# Autodesk Inventor assembly: 總組合圖
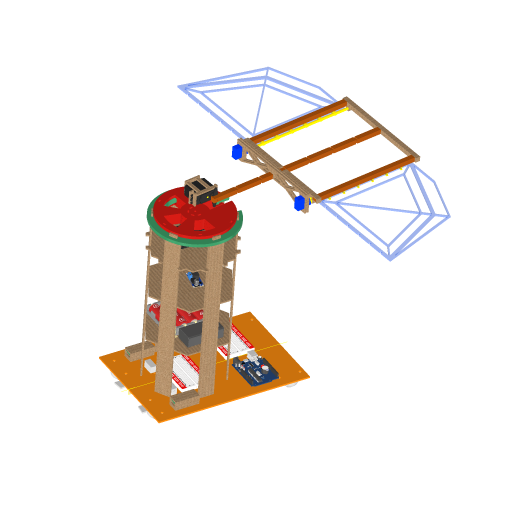
[picture p0: Inventor's stored thumbnail of the model, 512x512]
Saved by Autodesk Inventor 2024 (Build 280153000, 153)
## iProperties
Created: 2024-04-09
Document SubType Name: Assembly
Designer: USER
Mass: 1317.31 g
Surface Area: 9223.84 cm^2
Volume: 1282.93 cm^3
Author: 第26組
Title: 總組合圖
## Documents named in this file (26)
- C:\文件\機械工程實務\3D_CAD_Drawing\圖檔\DesignVer2_encoder_MG996\DesignVer_final.iam
- C:\文件\機械工程實務\3D_CAD_Drawing\圖檔\DesignVer2_encoder_MG996\cow_wheel.ipt
- C:\文件\機械工程實務\3D_CAD_Drawing\圖檔\DesignVer2_encoder_MG996\back_down_hold.ipt
- C:\文件\機械工程實務\3D_CAD_Drawing\圖檔\DesignVer2_encoder_MG996\middle_space.ipt
- C:\文件\機械工程實務\3D_CAD_Drawing\圖檔\DesignVer2_encoder_MG996\rolling_plate.ipt
- C:\文件\機械工程實務\3D_CAD_Drawing\圖檔\DesignVer2_encoder_MG996\rolling_plate_small.ipt
- C:\文件\機械工程實務\3D_CAD_Drawing\圖檔\DesignVer2_encoder_MG996\sail.iam
- C:\文件\機械工程實務\3D_CAD_Drawing\圖檔\DesignVer2_encoder_MG996\Base_final.ipt
- C:\文件\機械工程實務\3D_CAD_Drawing\圖檔\DesignVer2_encoder_MG996\[3DP]back_cir_hold_final.ipt
- C:\文件\機械工程實務\3D_CAD_Drawing\圖檔\DesignVer2_encoder_MG996\MG996R\MG_996R.iam
- C:\文件\機械工程實務\3D_CAD_Drawing\圖檔\DesignVer2_encoder_MG996\middle_space_3.ipt
- C:\文件\機械工程實務\3D_CAD_Drawing\圖檔\encoder\encoder.iam
- C:\文件\機械工程實務\3D_CAD_Drawing\圖檔\DesignVer2_encoder_MG996\Servo Motor SG90.ipt
- C:\文件\機械工程實務\3D_CAD_Drawing\圖檔\DesignVer2_encoder_MG996\final_circ_plate.ipt
- C:\文件\機械工程實務\3D_CAD_Drawing\圖檔\DesignVer2_encoder_MG996\final_side.ipt
- C:\文件\機械工程實務\3D_CAD_Drawing\圖檔\DesignVer2_encoder_MG996\final_side_hold.ipt
- C:\文件\機械工程實務\3D_CAD_Drawing\圖檔\DesignVer2_encoder_MG996\final_side_hold_2.ipt
- C:\文件\機械工程實務\3D_CAD_Drawing\圖檔\DesignVer2_encoder_MG996\final_side2.ipt
- C:\文件\機械工程實務\3D_CAD_Drawing\圖檔\DesignVer2_encoder_MG996\final_side_hold_3.ipt
- C:\文件\機械工程實務\3D_CAD_Drawing\圖檔\機電設備\18650電池盒\18650電池盒.ipt
- C:\文件\機械工程實務\3D_CAD_Drawing\圖檔\機電設備\Arduino板\Arduino板.iam
- C:\文件\機械工程實務\3D_CAD_Drawing\圖檔\機電設備\麵包板\麵包板.ipt
- C:\文件\機械工程實務\3D_CAD_Drawing\圖檔\機電設備\9V方型電池盒\9V方型電池盒.ipt
- C:\文件\機械工程實務\3D_CAD_Drawing\圖檔\DesignVer2_encoder_MG996\breaker.ipt
- C:\文件\機械工程實務\3D_CAD_Drawing\圖檔\機電設備\lm2596-dc-dc-buck-converter-module-2.snapshot.9\LM2596 DC-DC Buck Converter Module.iam
- LM2596 DC-DC Buck Converter Module.iam
## Components (45 placed, 24 different names)
1. cow_wheel:3 — 貼合:80, 貼合:81, 貼合:85
2. cow_wheel:4 — 貼合:75, 貼合:76, 貼合:77, 貼合:78, 貼合:79
3. back_down_hold:1 — 貼合:99, 貼合:100, 貼合:101, 貼合:102, 貼合:107
4. back_down_hold:2 — 齊平:14, 齊平:28, 貼合:92, 貼合:93, 貼合:94
5. back_down_hold:3 — 齊平:5, 貼合:47, 齊平:13, 貼合:90, 貼合:91, 貼合:108, 貼合:138, 貼合:139, 貼合:140
6. back_down_hold:4 — 貼合:87, 貼合:97, 貼合:98
7. back_down_hold:5 — 齊平:6, 貼合:46, 齊平:12, 貼合:48, 貼合:88, 貼合:89, 貼合:105
8. back_down_hold:6 — 齊平:5, 齊平:6, 貼合:95, 貼合:96, 貼合:109
9. middle_space:1 — 齊平:13, 貼合:48, 齊平:14, 齊平:28, 貼合:182, 貼合:186
10. middle_space:2 — 貼合:46, 齊平:12, 貼合:47, 貼合:189
11. rolling_plate:1 — 貼合:55, 齊平:22, 齊平:23, 貼合:155
12. rolling_plate:2 — 貼合:56, 貼合:57, 齊平:24, 貼合:110
13. rolling_plate_small:1 — 貼合:52, 齊平:16, 齊平:19, 貼合:56, 齊平:24, 貼合:142, 貼合:143, 貼合:144
14. rolling_plate_small:2 — 貼合:52, 貼合:53, 齊平:16, 齊平:17, 齊平:19, 齊平:20, 貼合:57
15. rolling_plate_small:3 — 貼合:53, 貼合:54, 齊平:17, 齊平:18, 齊平:20, 齊平:21, 貼合:156, 齊平:37
16. rolling_plate_small:4 — 貼合:54, 齊平:18, 齊平:21, 貼合:55, 齊平:22, 齊平:23
17. sail:1 [sub-assembly] — 角度:6, 貼合:181, 齊平:44
18. Base_final:1 — 貼合:75, 貼合:76, 貼合:77, 貼合:78, 貼合:79, 貼合:80, 貼合:81, 貼合:85, 貼合:87, 貼合:88, 貼合:89, 貼合:90, 貼合:91, 貼合:92, 貼合:93, 貼合:94, 貼合:95, 貼合:96, 貼合:97, 貼合:98, 貼合:99, 貼合:100, 貼合:101, 貼合:102, 貼合:105, 貼合:115, 貼合:116, 貼合:117, 貼合:118, 貼合:131, 貼合:134, 角度:2, 角度:4, 齊平:29, 貼合:145, 貼合:146, 貼合:147, 貼合:148, 貼合:149, 貼合:151, 貼合:152, 貼合:153, 角度:5, 齊平:33, 齊平:34, 齊平:35, 齊平:36, 貼合:154, 貼合:183, 貼合:184, 貼合:185
19. [3DP]back_cir_hold_final:1 — 貼合:107, 貼合:108, 貼合:109, 貼合:110, 貼合:142
20. cow_wheel:5 — 貼合:131, 貼合:145, 貼合:146, 貼合:147
21. cow_wheel:6 — 貼合:134, 貼合:148, 貼合:149
22. MG_996R:1 [sub-assembly] — 角度:2, 貼合:141, 貼合:143, 貼合:144, 角度:6
23. middle_space_3:1 — 貼合:138, 貼合:139, 貼合:140, 貼合:141
24. encoder:1 [sub-assembly] — 角度:3, 角度:4, 齊平:30, 貼合:151, 齊平:31, 貼合:154
25. encoder:2 [sub-assembly] — 角度:3, 齊平:29, 齊平:30, 齊平:31, 貼合:152
26. Servo Motor SG90:1 — 齊平:32, 貼合:153, 角度:5, 齊平:33, 齊平:34, 貼合:188
27. Servo Motor SG90:2 — 齊平:32, 齊平:35, 齊平:36, 貼合:187
28. final_circ_plate:1 — 貼合:155, 貼合:156, 齊平:37, 貼合:157, 貼合:158, 貼合:159, 貼合:160, 貼合:161, 貼合:164, 貼合:165, 貼合:166, 貼合:167, 貼合:168, 貼合:169, 貼合:170, 貼合:173, 貼合:174, 貼合:175
29. MG_996R:2 [sub-assembly] — 貼合:157, 貼合:171, 貼合:172, 貼合:181, 齊平:44
30. final_side:1 — 貼合:164, 貼合:165, 貼合:169, 貼合:176, 齊平:39, 貼合:177
31. final_side:2 — 貼合:166, 貼合:167, 貼合:168
32. final_side_hold:1 — 貼合:176, 齊平:39, 貼合:177, 貼合:178, 齊平:41
33. final_side_hold_2:1 — 貼合:173, 貼合:174, 貼合:175, 齊平:40, 齊平:42, 貼合:180
34. final_side2:1 — 貼合:158, 貼合:159, 貼合:170, 齊平:38
35. final_side2:2 — 貼合:160, 貼合:161, 齊平:38, 貼合:171, 貼合:172
36. final_side_hold_3:1 — 齊平:40, 齊平:43, 貼合:180
37. final_side_hold_3:2 — 貼合:178, 齊平:41, 齊平:42, 齊平:43
38. 18650電池盒:1 — 貼合:182, 齊平:45
39. Arduino板:1 [sub-assembly] — 貼合:183
40. 麵包板:1 — 貼合:184
41. 麵包板:2 — 貼合:185
42. 9V方型電池盒:1 — 貼合:186, 齊平:45
43. breaker:1 — 貼合:187
44. breaker:2 — 貼合:188
45. LM2596 DC-DC Buck Converter Module:1 [sub-assembly] — 貼合:189
## Relationships (131: Mate 94, Flush 32, Angle 5)
- 齊平:5 [Flush]: back_down_hold:3 ↔ back_down_hold:6
- 齊平:6 [Flush]: back_down_hold:5 ↔ back_down_hold:6
- 貼合:46 [Mate]: back_down_hold:5 ↔ middle_space:2
- 齊平:12 [Flush]: back_down_hold:5 ↔ middle_space:2
- 貼合:47 [Mate]: back_down_hold:3 ↔ middle_space:2
- 齊平:13 [Flush]: back_down_hold:3 ↔ middle_space:1
- 貼合:48 [Mate]: back_down_hold:5 ↔ middle_space:1
- 齊平:14 [Flush]: back_down_hold:2 ↔ middle_space:1
- 貼合:52 [Mate]: rolling_plate_small:1 ↔ rolling_plate_small:2
- 貼合:53 [Mate]: rolling_plate_small:2 ↔ rolling_plate_small:3
- 貼合:54 [Mate]: rolling_plate_small:3 ↔ rolling_plate_small:4
- 齊平:16 [Flush]: rolling_plate_small:1 ↔ rolling_plate_small:2
- 齊平:17 [Flush]: rolling_plate_small:2 ↔ rolling_plate_small:3
- 齊平:18 [Flush]: rolling_plate_small:3 ↔ rolling_plate_small:4
- 齊平:19 [Flush]: rolling_plate_small:1 ↔ rolling_plate_small:2
- 齊平:20 [Flush]: rolling_plate_small:2 ↔ rolling_plate_small:3
- 齊平:21 [Flush]: rolling_plate_small:3 ↔ rolling_plate_small:4
- 貼合:55 [Mate]: rolling_plate:1 ↔ rolling_plate_small:4
- 齊平:22 [Flush]: rolling_plate:1 ↔ rolling_plate_small:4
- 齊平:23 [Flush]: rolling_plate:1 ↔ rolling_plate_small:4
- 貼合:56 [Mate]: rolling_plate:2 ↔ rolling_plate_small:1
- 貼合:57 [Mate]: rolling_plate:2 ↔ rolling_plate_small:2
- 齊平:24 [Flush]: rolling_plate:2 ↔ rolling_plate_small:1
- 齊平:28 [Flush]: back_down_hold:2 ↔ middle_space:1
- 貼合:75 [Mate]: cow_wheel:4 ↔ Base_final:1
- 貼合:76 [Mate]: cow_wheel:4 ↔ Base_final:1
- 貼合:77 [Mate]: cow_wheel:4 ↔ Base_final:1
- 貼合:78 [Mate]: cow_wheel:4 ↔ Base_final:1
- 貼合:79 [Mate]: cow_wheel:4 ↔ Base_final:1
- 貼合:80 [Mate]: cow_wheel:3 ↔ Base_final:1
- 貼合:81 [Mate]: cow_wheel:3 ↔ Base_final:1
- 貼合:85 [Mate]: cow_wheel:3 ↔ Base_final:1
- 貼合:87 [Mate]: back_down_hold:4 ↔ Base_final:1
- 貼合:88 [Mate]: back_down_hold:5 ↔ Base_final:1
- 貼合:89 [Mate]: back_down_hold:5 ↔ Base_final:1
- 貼合:90 [Mate]: back_down_hold:3 ↔ Base_final:1
- 貼合:91 [Mate]: back_down_hold:3 ↔ Base_final:1
- 貼合:92 [Mate]: back_down_hold:2 ↔ Base_final:1
- 貼合:93 [Mate]: back_down_hold:2 ↔ Base_final:1
- 貼合:94 [Mate]: back_down_hold:2 ↔ Base_final:1
- 貼合:95 [Mate]: back_down_hold:6 ↔ Base_final:1
- 貼合:96 [Mate]: back_down_hold:6 ↔ Base_final:1
- 貼合:97 [Mate]: back_down_hold:4 ↔ Base_final:1
- 貼合:98 [Mate]: back_down_hold:4 ↔ Base_final:1
- 貼合:99 [Mate]: back_down_hold:1 ↔ Base_final:1
- 貼合:100 [Mate]: back_down_hold:1 ↔ Base_final:1
- 貼合:101 [Mate]: back_down_hold:1 ↔ Base_final:1
- 貼合:102 [Mate]: back_down_hold:1 ↔ Base_final:1
- 貼合:105 [Mate]: back_down_hold:5 ↔ Base_final:1
- 貼合:107 [Mate]: back_down_hold:1 ↔ [3DP]back_cir_hold_final:1
- 貼合:108 [Mate]: back_down_hold:3 ↔ [3DP]back_cir_hold_final:1
- 貼合:109 [Mate]: back_down_hold:6 ↔ [3DP]back_cir_hold_final:1
- 貼合:110 [Mate] (0.5 mm): rolling_plate:2 ↔ [3DP]back_cir_hold_final:1
- 貼合:115 [Mate]: Base_final:1
- 貼合:116 [Mate]: Base_final:1
- 貼合:117 [Mate]: Base_final:1
- 貼合:118 [Mate]: Base_final:1
- 貼合:119 [Mate]
- 貼合:120 [Mate]
- 貼合:131 [Mate]: Base_final:1 ↔ cow_wheel:5
- 貼合:134 [Mate]: Base_final:1 ↔ cow_wheel:6
- 角度:2 [Angle] (0 deg): Base_final:1 ↔ MG_996R:1
- 貼合:138 [Mate]: back_down_hold:3 ↔ middle_space_3:1
- 貼合:139 [Mate]: back_down_hold:3 ↔ middle_space_3:1
- 貼合:140 [Mate]: back_down_hold:3 ↔ middle_space_3:1
- 貼合:141 [Mate]: MG_996R:1 ↔ middle_space_3:1
- 貼合:142 [Mate]: rolling_plate_small:1 ↔ [3DP]back_cir_hold_final:1
- 貼合:143 [Mate]: rolling_plate_small:1 ↔ MG_996R:1
- 貼合:144 [Mate]: rolling_plate_small:1 ↔ MG_996R:1
- 角度:3 [Angle] (0 deg): encoder:1 ↔ encoder:2
- 角度:4 [Angle] (0 deg): Base_final:1 ↔ encoder:1
- 齊平:29 [Flush] (-12 mm): Base_final:1 ↔ encoder:2
- 齊平:30 [Flush]: encoder:1 ↔ encoder:2
- 貼合:145 [Mate]: Base_final:1 ↔ cow_wheel:5
- 貼合:146 [Mate]: Base_final:1 ↔ cow_wheel:5
- 貼合:147 [Mate]: Base_final:1 ↔ cow_wheel:5
- 貼合:148 [Mate]: Base_final:1 ↔ cow_wheel:6
- 貼合:149 [Mate]: Base_final:1 ↔ cow_wheel:6
- 貼合:151 [Mate] (0.1 mm): Base_final:1 ↔ encoder:1
- 齊平:31 [Flush]: encoder:1 ↔ encoder:2
- 貼合:152 [Mate] (0.1 mm): Base_final:1 ↔ encoder:2
- 齊平:32 [Flush]: Servo Motor SG90:1 ↔ Servo Motor SG90:2
- 貼合:153 [Mate]: Base_final:1 ↔ Servo Motor SG90:1
- 角度:5 [Angle] (0 deg): Base_final:1 ↔ Servo Motor SG90:1
- 齊平:33 [Flush] (55 mm): Base_final:1 ↔ Servo Motor SG90:1
- 齊平:34 [Flush] (55 mm): Base_final:1 ↔ Servo Motor SG90:1
- 齊平:35 [Flush] (55 mm): Base_final:1 ↔ Servo Motor SG90:2
- 齊平:36 [Flush] (55 mm): Base_final:1 ↔ Servo Motor SG90:2
- 貼合:154 [Mate] (0.1 mm): Base_final:1 ↔ encoder:1
- 貼合:155 [Mate]: rolling_plate:1 ↔ final_circ_plate:1
- 貼合:156 [Mate]: rolling_plate_small:3 ↔ final_circ_plate:1
- 齊平:37 [Flush]: rolling_plate_small:3 ↔ final_circ_plate:1
- 貼合:157 [Mate]: final_circ_plate:1 ↔ MG_996R:2
- 貼合:158 [Mate]: final_circ_plate:1 ↔ final_side2:1
- 貼合:159 [Mate]: final_circ_plate:1 ↔ final_side2:1
- 貼合:160 [Mate]: final_circ_plate:1 ↔ final_side2:2
- 貼合:161 [Mate]: final_circ_plate:1 ↔ final_side2:2
- 貼合:164 [Mate]: final_circ_plate:1 ↔ final_side:1
- 貼合:165 [Mate]: final_circ_plate:1 ↔ final_side:1
- 貼合:166 [Mate]: final_circ_plate:1 ↔ final_side:2
- 貼合:167 [Mate]: final_circ_plate:1 ↔ final_side:2
- 貼合:168 [Mate]: final_circ_plate:1 ↔ final_side:2
- 貼合:169 [Mate]: final_circ_plate:1 ↔ final_side:1
- 貼合:170 [Mate]: final_circ_plate:1 ↔ final_side2:1
- 齊平:38 [Flush]: final_side2:1 ↔ final_side2:2
- 貼合:171 [Mate]: MG_996R:2 ↔ final_side2:2
- 貼合:172 [Mate]: MG_996R:2 ↔ final_side2:2
- 貼合:173 [Mate]: final_circ_plate:1 ↔ final_side_hold_2:1
- 貼合:174 [Mate]: final_circ_plate:1 ↔ final_side_hold_2:1
- 貼合:175 [Mate]: final_circ_plate:1 ↔ final_side_hold_2:1
- 貼合:176 [Mate]: final_side:1 ↔ final_side_hold:1
- 齊平:39 [Flush]: final_side:1 ↔ final_side_hold:1
- 貼合:177 [Mate]: final_side:1 ↔ final_side_hold:1
- 齊平:40 [Flush]: final_side_hold_2:1 ↔ final_side_hold_3:1
- 貼合:178 [Mate]: final_side_hold:1 ↔ final_side_hold_3:2
- 齊平:41 [Flush]: final_side_hold:1 ↔ final_side_hold_3:2
- 齊平:42 [Flush]: final_side_hold_2:1 ↔ final_side_hold_3:2
- 齊平:43 [Flush]: final_side_hold_3:1 ↔ final_side_hold_3:2
- 貼合:180 [Mate]: final_side_hold_2:1 ↔ final_side_hold_3:1
- 角度:6 [Angle] (0 deg): sail:1 ↔ MG_996R:1
- 貼合:181 [Mate]: sail:1 ↔ MG_996R:2
- 齊平:44 [Flush]: sail:1 ↔ MG_996R:2
- 貼合:182 [Mate]: middle_space:1 ↔ 18650電池盒:1
- 貼合:183 [Mate]: Base_final:1 ↔ Arduino板:1
- 貼合:184 [Mate]: Base_final:1 ↔ 麵包板:1
- 貼合:185 [Mate]: Base_final:1 ↔ 麵包板:2
- 貼合:186 [Mate]: middle_space:1 ↔ 9V方型電池盒:1
- 齊平:45 [Flush]: 18650電池盒:1 ↔ 9V方型電池盒:1
- 貼合:187 [Mate]: Servo Motor SG90:2 ↔ breaker:1
- 貼合:188 [Mate]: Servo Motor SG90:1 ↔ breaker:2
- 貼合:189 [Mate]: middle_space:2 ↔ LM2596 DC-DC Buck Converter Module:1
